# Autodesk Inventor assembly: Frame
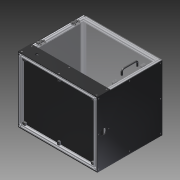
[picture p0: Inventor's stored thumbnail of the model, 180x180]
Saved by Autodesk Inventor 2015 SP1 (Build 190203100, 203)
## iProperties
Created: 2014-08-02
Part Number: Frame
Document SubType Name: Assembly
Designer: Jack
Mass: 3721.39 g
Surface Area: 12751.2 cm^2
Volume: 1360.83 cm^3
Density: 2.73465 g/cm^3
Author: Jack
Title: Frame
## Documents named in this file (29)
- C:\Users\Jack\ownCloud\Projects\CoreXY\InventorModel\Frame\Frame.iam
- C:\Users\Jack\ownCloud\Projects\CoreXY\InventorModel\Frame\FrameFrontBack.ipt
- C:\Users\Jack\ownCloud\Projects\CoreXY\InventorModel\Frame\FrameSide.ipt
- C:\Users\Jack\ownCloud\Projects\CoreXY\InventorModel\Frame\FrameUpright.ipt
- C:\Users\Jack\ownCloud\Projects\CoreXY\InventorModel\Hardware\Bolts\BlindExtrusionScrew\BlindExtrusionScrew5\M5x20BlindScrew.ipt
- C:\Users\Jack\ownCloud\Projects\CoreXY\InventorModel\Frame\FrameExtruderVerticalSupport.ipt
- C:\Users\Jack\ownCloud\Projects\CoreXY\InventorModel\Enclosure\EnclosurePanelBack.ipt
- C:\Users\Jack\ownCloud\Projects\CoreXY\InventorModel\Enclosure\EnclosurePanelBottomFront.ipt
- C:\Users\Jack\ownCloud\Projects\CoreXY\InventorModel\Enclosure\ElectronicsLowerPanel.ipt
- C:\Users\Jack\ownCloud\Projects\CoreXY\InventorModel\Enclosure\EnclosureDoorFront.ipt
- C:\Users\Jack\ownCloud\Projects\CoreXY\InventorModel\Hardware\PanelMounts\HCBR5.ipt
- C:\Users\Jack\ownCloud\Projects\CoreXY\InventorModel\Hardware\Bolts\SHCS\SHCS5\SHCS5x15.ipt
- C:\Users\Jack\ownCloud\Projects\CoreXY\InventorModel\Hardware\Hinges\HingeSHHPSK5-2\SHHPSK5_2.iam
- C:\Users\Jack\ownCloud\Projects\CoreXY\InventorModel\Hardware\FrameBrace\FrameBraceHBLFSN5-4.ipt
- C:\Users\Jack\ownCloud\Projects\CoreXY\InventorModel\Enclosure\ElectronicsTopPanel.ipt
- C:\Users\Jack\ownCloud\Projects\CoreXY\InventorModel\Hardware\Handles\HandleUWANGF100-5.ipt
- C:\Users\Jack\ownCloud\Projects\CoreXY\InventorModel\Hardware\Bolts\SHCS\SHCS4\SHCS4x10.ipt
- C:\Users\Jack\ownCloud\Projects\CoreXY\InventorModel\Hardware\Nuts\ExtrusionNuts\ExtrusionNutHNTT5-4.ipt
- C:\Users\Jack\ownCloud\Projects\CoreXY\InventorModel\Hardware\BoltWashers\BoltWasher5\BoltWasher5x8.iam
- C:\Users\Jack\ownCloud\Projects\CoreXY\InventorModel\Hardware\Nuts\Nut4.ipt
- C:\Users\Jack\ownCloud\Projects\CoreXY\InventorModel\Hardware\BoltWashers\BoltWasher5\BoltWasher5x10.iam
- C:\Users\Jack\ownCloud\Projects\CoreXY\InventorModel\Hardware\Nuts\ExtrusionNuts\ExtrusionNutLockHNTR5-4.ipt
- C:\Users\Jack\ownCloud\Projects\CoreXY\InventorModel\Hardware\Bolts\FHS\FHS4\FHS4x10.ipt
- C:\Users\Jack\ownCloud\Projects\CoreXY\InventorModel\Enclosure\EnclosurePanelLeft.ipt
- C:\Users\Jack\ownCloud\Projects\CoreXY\InventorModel\Enclosure\EnclosurePanelRight.ipt
- C:\Users\Jack\ownCloud\Projects\CoreXY\InventorModel\Hardware\Bolts\SHCS\SHCS5\SHCS5x16.ipt
- C:\Users\Jack\ownCloud\Projects\CoreXY\InventorModel\Hardware\Catches\CatchMagnetHMEN5-5\HMEN5_5_dps.ipt
- C:\Users\Jack\ownCloud\Projects\CoreXY\InventorModel\Hardware\Catches\CatchMagnetHMEN5-5\HMEN5_5_magnet.ipt
- C:\Users\Jack\ownCloud\Projects\CoreXY\InventorModel\Hardware\BoltWashers\BoltWasher4\BoltWasher4x8.iam
## Components (204 placed, 28 different names)
1. SHCS5x16:1 — Mate:400, Mate:403
2. SHCS5x16:2 — Mate:401, Mate:402
3. FrameSide:6 — Mate:66, Flush:32, Flush:33, Mate:136, Mate:146, Flush:74, Mate:148, Flush:75, Mate:181, Mate:183, Mate:211, Angle:2, Angle:21, Mate:328
4. FrameSide:5 — Mate:64, Flush:28, Flush:30, Mate:138, Mate:151, Flush:78, Mate:152, Flush:79, Mate:180, Mate:184, Mate:214, Angle:3, Angle:36, Angle:51, Mate:398
5. FrameSide:4 — Mate:52, Flush:23, Flush:25, Flush:26, Mate:84, Flush:51, Mate:86, Flush:52, Mate:94, Angle:35, Angle:50, Mate:397
6. FrameSide:3 — Mate:51, Flush:22, Flush:27, Mate:88, Flush:53, Mate:90, Flush:54, Angle:20, Mate:329
7. FrameSide:1 — Mate:1, Flush:1, Flush:2, Mate:3, Flush:5, Flush:6, Mate:18, Mate:22, Angle:25, Mate:342, Flush:114, Mate:363
8. FrameSide:2 — Mate:6, Flush:11, Flush:12, Mate:7, Mate:25, Mate:26, Mate:343, Flush:113, Angle:40, Mate:379
9. FrameExtruderVerticalSupport:1 — Mate:67, Flush:37, Mate:69, Mate:123, Flush:64, Mate:176, Mate:178, Mate:231, Angle:11
10. FrameExtruderVerticalSupport:2 — Mate:68, Flush:36, Mate:70, Mate:124, Flush:65, Mate:177, Mate:179, Mate:230, Angle:12
11. FrameUpright:1 — Mate:1, Flush:1, Flush:2, Mate:2, Flush:3, Flush:4, Mate:42, Mate:43, Mate:48, Mate:49, Mate:53, Flush:21, Flush:22, Mate:61, Mate:62, Mate:65, Mate:66, Flush:33, Flush:34, Mate:70, Flush:69, Mate:132, Mate:191, Mate:199, Mate:229, Angle:10, Angle:22, Angle:23, Angle:24, Mate:325, Mate:326, Mate:327, Angle:47, Angle:48, Angle:49, Mate:390, Mate:391, Mate:392
12. FrameUpright:2 — Mate:3, Flush:5, Flush:6, Mate:5, Flush:9, Flush:10, Mate:12, Mate:13, Mate:19, Mate:21, Mate:36, Mate:37, Mate:50, Mate:51, Mate:54, Mate:55, Mate:56, Flush:61, Mate:112, Mate:113, Mate:114, Mate:115, Mate:116, Mate:117, Mate:137, Flush:71, Mate:192, Mate:193, Mate:210, Angle:1, Angle:13, Angle:14, Angle:15, Angle:16, Mate:252, Mate:253, Mate:254, Mate:255, Mate:281, Angle:17, Angle:18, Mate:323, Angle:19, Mate:324, Angle:26, Angle:27, Mate:338, Mate:339, Flush:115
13. FrameUpright:3 — Mate:7, Mate:8, Flush:13, Mate:38, Mate:39, Mate:46, Mate:47, Mate:52, Flush:23, Flush:24, Mate:57, Mate:58, Mate:63, Mate:64, Flush:28, Flush:29, Mate:139, Flush:72, Mate:194, Mate:195, Mate:227, Angle:8, Angle:28, Angle:29, Mate:336, Mate:337, Flush:116, Mate:365, Angle:32, Mate:367, Mate:369, Angle:33, Angle:34, Mate:404, Flush:136, Mate:405, Flush:137, Mate:410, Angle:52, Mate:411, Mate:414, Angle:53, Mate:417, Mate:420, Mate:421, Mate:422, Mate:423
14. FrameUpright:4 — Mate:4, Flush:7, Flush:8, Mate:6, Flush:11, Flush:12, Mate:40, Mate:41, Mate:44, Mate:45, Mate:59, Mate:60, Mate:69, Mate:134, Flush:70, Mate:190, Mate:198, Mate:228, Angle:9, Mate:373, Angle:37, Mate:375, Angle:38, Mate:377, Angle:39, Flush:135, Mate:381, Angle:41, Angle:43, Angle:44, Mate:395, Mate:396
15. FrameFrontBack:3 — Mate:50, Flush:24, Flush:25, Mate:54, Flush:35, Flush:39, Mate:85, Mate:91, Mate:92, Flush:55, Angle:31, Mate:341
16. FrameFrontBack:6 — Mate:65, Flush:34, Mate:67, Mate:68, Flush:36, Flush:37, Mate:122, Mate:125, Mate:130, Mate:135, Mate:149, Mate:154, Mate:186, Mate:187, Mate:196, Mate:197, Mate:216, Angle:4, Mate:219, Angle:5, Mate:222, Angle:6, Mate:224, Angle:7, Angle:45, Mate:393
17. FrameFrontBack:5 — Mate:63, Flush:29, Flush:30, Flush:32, Flush:35, Mate:73, Mate:118, Mate:145, Flush:73, Mate:147, Mate:153, Mate:182, Mate:185, Angle:30, Mate:340, Mate:407
18. FrameFrontBack:4 — Mate:53, Flush:21, Flush:26, Flush:27, Flush:44, Mate:87, Mate:89, Mate:93, Flush:56, Angle:46, Mate:394
19. FrameFrontBack:1 — Mate:2, Flush:3, Flush:4, Mate:4, Flush:7, Flush:8, Mate:23, Mate:24, Mate:76, Mate:188, Mate:189, Angle:42, Mate:399
20. FrameFrontBack:2 — Mate:5, Flush:9, Flush:10, Mate:8, Flush:13, Flush:20, Mate:20, Mate:27, Flush:63, Mate:406
21. EnclosurePanelLeft:1 — Mate:342, Flush:114, Flush:115, Mate:344, Mate:353, Mate:354, Mate:355, Flush:117, Flush:118, Flush:119, Flush:120, Mate:356, Flush:121, Mate:357, Flush:122, Mate:358, Flush:123, Mate:359, Flush:124, Mate:360, Flush:125
22. EnclosurePanelRight:1 — Mate:343, Flush:113, Flush:116, Mate:345, Mate:346, Mate:347, Mate:348, Mate:349, Mate:350, Mate:351, Mate:352, Flush:126, Flush:127, Flush:128, Mate:361, Flush:129, Flush:130, Flush:131, Flush:132, Flush:133, Flush:134
23. HandleUWANGF100-5:1 — Mate:171, Mate:172, Mate:173
24. EnclosurePanelBack:1 — Mate:76, Flush:44, Mate:298, Mate:299, Mate:300, Mate:301, Mate:302, Mate:303, Mate:304, Mate:305, Flush:96, Flush:97, Flush:98, Flush:99, Flush:100, Flush:101, Flush:102, Flush:103, Mate:306, Flush:104, Flush:135
25. EnclosurePanelBottomFront:1 — Mate:73, Flush:39, Flush:61, Mate:309, Flush:107, Mate:310, Flush:108, Mate:311, Flush:109, Mate:312, Flush:110, Mate:313, Mate:314, Flush:111, Flush:112
26. EnclosureDoorFront:1 — Mate:120, Mate:121, Mate:171, Mate:172, Mate:173, Mate:174, Mate:175, Mate:264, Mate:265, Mate:266, Mate:267, Mate:268, Mate:269, Mate:270, Mate:271, Mate:400, Mate:401, Mate:402, Mate:403, Mate:408, Mate:409, Flush:138, Flush:139, Flush:140, Flush:141
27. ExtrusionNutHNTT5-4:20 — Mate:421, Mate:423
28. ExtrusionNutHNTT5-4:19 — Mate:420, Mate:422
29. BoltWasher4x8:4 [sub-assembly] — Mate:425, Tangent:4
30. BoltWasher4x8:3 [sub-assembly] — Mate:424, Tangent:3
31. HMEN5_5_dps:1 — Mate:408, Flush:139, Flush:141
32. HMEN5_5_dps:2 — Mate:409, Flush:138, Flush:140
33. BoltWasher4x8:2 [sub-assembly] — Mate:415, Mate:416, Tangent:2
34. ExtrusionNutHNTT5-4:17 — Mate:410, Angle:52, Mate:411, Mate:412
35. ExtrusionNutHNTT5-4:18 — Mate:414, Angle:53, Mate:415, Mate:417
36. HMEN5_5_magnet:2 — Mate:405, Flush:137, Mate:406, Tangent:1, Mate:413, Mate:416, Tangent:2
37. BoltWasher4x8:1 [sub-assembly] — Mate:412, Tangent:1, Mate:413
38. HMEN5_5_magnet:1 — Mate:404, Flush:136, Mate:407, Mate:424, Mate:425, Tangent:3, Tangent:4
39. ExtrusionNutLockHNTR5-4:26 — Mate:382, Angle:44, Mate:395
40. ExtrusionNutLockHNTR5-4:27 — Mate:383, Angle:43, Mate:396
41. ExtrusionNutLockHNTR5-4:28 — Mate:384, Angle:42, Mate:399
42. ExtrusionNutLockHNTR5-4:29 — Mate:385, Angle:49, Mate:390
43. ExtrusionNutLockHNTR5-4:30 — Mate:386, Angle:48, Mate:391
44. ExtrusionNutLockHNTR5-4:31 — Mate:387, Angle:47, Mate:392
45. ExtrusionNutLockHNTR5-4:32 — Mate:388, Angle:46, Mate:394
46. ExtrusionNutLockHNTR5-4:33 — Mate:389, Angle:45, Mate:393
47. ExtrusionNutLockHNTR5-4:25 — Mate:380, Mate:381, Angle:41
48. FHS4x10:22 — Mate:303, Flush:98, Mate:383
49. FHS4x10:25 — Mate:306, Flush:104, Mate:384
50. FHS4x10:23 — Mate:304, Flush:97, Mate:382
51. FHS4x10:24 — Mate:305, Flush:96, Mate:380
52. FHS4x10:21 — Mate:302, Flush:99, Mate:389
53. FHS4x10:20 — Mate:301, Flush:100, Mate:388
54. FHS4x10:19 — Mate:300, Flush:101, Mate:387
55. FHS4x10:18 — Mate:299, Flush:102, Mate:386
56. FHS4x10:17 — Mate:298, Flush:103, Mate:385
57. ExtrusionNutLockHNTR5-4:1 — Mate:281, Angle:17, Mate:362
58. ExtrusionNutLockHNTR5-4:2 — Mate:315, Angle:18, Mate:323
59. ExtrusionNutLockHNTR5-4:3 — Mate:316, Angle:19, Mate:324
60. ExtrusionNutLockHNTR5-4:4 — Mate:317, Angle:20, Mate:329
61. ExtrusionNutLockHNTR5-4:5 — Mate:318, Angle:21, Mate:328
62. ExtrusionNutLockHNTR5-4:6 — Mate:319, Angle:22, Mate:327
63. ExtrusionNutLockHNTR5-4:7 — Mate:320, Angle:23, Mate:326
64. ExtrusionNutLockHNTR5-4:8 — Mate:321, Angle:24, Mate:325
65. ExtrusionNutLockHNTR5-4:9 — Mate:322, Angle:25, Mate:363
66. FHS4x10:26 — Mate:318, Mate:360, Flush:125
67. FHS4x10:6 — Mate:316, Mate:355, Flush:120
68. FHS4x10:3 — Mate:319, Mate:358, Flush:123
69. FHS4x10:7 — Mate:320, Mate:357, Flush:122
70. FHS4x10:5 — Mate:321, Mate:356, Flush:121
71. FHS4x10:2 — Mate:322, Mate:344, Flush:117
72. FHS4x10:1 — Mate:353, Flush:118, Mate:362
73. FHS4x10:8 — Mate:315, Mate:354, Flush:119
74. FHS4x10:4 — Mate:317, Mate:359, Flush:124
75. ExtrusionNutLockHNTR5-4:16 — Mate:364, Mate:365, Angle:32
76. ExtrusionNutLockHNTR5-4:17 — Mate:366, Mate:367, Angle:34
77. ExtrusionNutLockHNTR5-4:18 — Mate:368, Mate:369, Angle:33
78. ExtrusionNutLockHNTR5-4:19 — Mate:370, Angle:35, Angle:50, Mate:397
79. ExtrusionNutLockHNTR5-4:20 — Mate:371, Angle:36, Angle:51, Mate:398
80. ExtrusionNutLockHNTR5-4:21 — Mate:372, Mate:373, Angle:37
81. ExtrusionNutLockHNTR5-4:22 — Mate:374, Mate:375, Angle:38
82. ExtrusionNutLockHNTR5-4:23 — Mate:376, Mate:377, Angle:39
83. ExtrusionNutLockHNTR5-4:24 — Mate:378, Angle:40, Mate:379
84. FHS4x10:27 — Mate:349, Flush:134, Mate:371
85. FHS4x10:14 — Mate:348, Flush:133, Mate:370
86. FHS4x10:16 — Mate:347, Flush:128, Mate:364
87. FHS4x10:11 — Mate:346, Flush:127, Mate:366
88. FHS4x10:10 — Mate:345, Flush:126, Mate:368
89. FHS4x10:9 — Mate:352, Flush:130, Mate:376
90. FHS4x10:15 — Mate:361, Flush:129, Mate:378
91. FHS4x10:12 — Mate:351, Flush:131, Mate:374
92. FHS4x10:13 — Mate:350, Flush:132, Mate:372
93. ExtrusionNutLockHNTR5-4:10 — Mate:330, Angle:27, Mate:338
94. ExtrusionNutLockHNTR5-4:11 — Mate:331, Angle:26, Mate:339
95. ExtrusionNutLockHNTR5-4:12 — Mate:332, Angle:31, Mate:341
96. ExtrusionNutLockHNTR5-4:13 — Mate:333, Angle:30, Mate:340
97. ExtrusionNutLockHNTR5-4:14 — Mate:334, Angle:28, Mate:336
98. ExtrusionNutLockHNTR5-4:15 — Mate:335, Angle:29, Mate:337
99. FHS4x10:28 — Mate:309, Flush:107, Mate:331
100. FHS4x10:29 — Mate:310, Flush:108, Mate:330
101. FHS4x10:30 — Mate:311, Flush:109, Mate:332
102. FHS4x10:31 — Mate:312, Flush:110, Mate:333
103. FHS4x10:32 — Mate:313, Flush:112, Mate:335
104. FHS4x10:33 — Mate:314, Flush:111, Mate:334
105. M5x20BlindScrew:17 — Mate:176, Mate:189
106. M5x20BlindScrew:18 — Mate:177, Mate:188
107. M5x20BlindScrew:19 — Mate:178, Mate:187
108. M5x20BlindScrew:20 — Mate:179, Mate:186
109. M5x20BlindScrew:21 — Mate:180, Mate:190
110. M5x20BlindScrew:22 — Mate:181, Mate:191
111. M5x20BlindScrew:23 — Mate:182, Mate:192
112. M5x20BlindScrew:24 — Mate:183, Mate:193
113. M5x20BlindScrew:25 — Mate:184, Mate:194
114. M5x20BlindScrew:26 — Mate:185, Mate:195
115. M5x20BlindScrew:27 — Mate:196, Mate:199
116. M5x20BlindScrew:28 — Mate:197, Mate:198
117. M5x20BlindScrew:1 — Mate:22, Mate:43
118. M5x20BlindScrew:2 — Mate:24, Mate:40
119. M5x20BlindScrew:3 — Mate:49, Mate:61
120. M5x20BlindScrew:4 — Mate:36, Mate:55
121. M5x20BlindScrew:5 — Mate:48, Mate:62
122. M5x20BlindScrew:6 — Mate:44, Mate:60
123. M5x20BlindScrew:7 — Mate:46, Mate:58
124. M5x20BlindScrew:8 — Mate:27, Mate:38
125. M5x20BlindScrew:9 — Mate:26, Mate:39
126. M5x20BlindScrew:10 — Mate:25, Mate:41
127. M5x20BlindScrew:11 — Mate:20, Mate:21
128. M5x20BlindScrew:12 — Mate:23, Mate:42
129. M5x20BlindScrew:13 — Mate:37, Mate:56
130. M5x20BlindScrew:14 — Mate:45, Mate:59
131. M5x20BlindScrew:15 — Mate:47, Mate:57
132. M5x20BlindScrew:16 — Mate:18, Mate:19
133. ExtrusionNutHNTT5-4:1 — Mate:208, Mate:211, Angle:2
134. ExtrusionNutHNTT5-4:2 — Mate:209, Mate:210, Angle:1
135. ExtrusionNutHNTT5-4:3 — Mate:212, Mate:214, Angle:3
136. ExtrusionNutHNTT5-4:4 — Mate:213, Mate:227, Angle:8
137. ExtrusionNutHNTT5-4:5 — Mate:215, Mate:216, Angle:4
138. ExtrusionNutHNTT5-4:6 — Mate:217, Mate:228, Angle:9
139. ExtrusionNutHNTT5-4:7 — Mate:218, Mate:219, Angle:5
140. ExtrusionNutHNTT5-4:8 — Mate:220, Mate:229, Angle:10
141. ExtrusionNutHNTT5-4:9 — Mate:221, Mate:222, Angle:6
142. ExtrusionNutHNTT5-4:10 — Mate:223, Mate:224, Angle:7
143. ExtrusionNutHNTT5-4:11 — Mate:225, Mate:230, Angle:12
144. ExtrusionNutHNTT5-4:12 — Mate:226, Mate:231, Angle:11
145. SHCS4x10:3 — Mate:201, Mate:202
146. SHCS4x10:12 — Mate:200, Mate:203
147. SHCS4x10:9 — Mate:232, Mate:244
148. SHCS4x10:11 — Mate:233, Mate:247
149. SHCS4x10:6 — Mate:235, Mate:243
150. SHCS4x10:8 — Mate:234, Mate:246
151. SHCS4x10:7 — Mate:236, Mate:245
152. SHCS4x10:1 — Mate:237, Mate:242
153. SHCS4x10:2 — Mate:238, Mate:241
154. SHCS4x10:5 — Mate:239, Mate:240
155. SHCS4x10:4 — Mate:205, Mate:206
156. SHCS4x10:10 — Mate:204, Mate:207
157. FrameBraceHBLFSN5-4:1 — Mate:122, Mate:123, Flush:64, Mate:223, Mate:226, Mate:236, Mate:237, Mate:242, Mate:245
158. FrameBraceHBLFSN5-4:2 — Mate:124, Flush:65, Mate:125, Mate:221, Mate:225, Mate:234, Mate:235, Mate:243, Mate:246
159. FrameBraceHBLFSN5-4:5 — Mate:130, Flush:69, Mate:132, Mate:218, Mate:220, Mate:232, Mate:233, Mate:244, Mate:247
160. FrameBraceHBLFSN5-4:7 — Mate:134, Mate:135, Flush:70, Mate:215, Mate:217, Mate:238, Mate:239, Mate:240, Mate:241
161. FrameBraceHBLFSN5-4:8 — Mate:136, Mate:137, Flush:71, Mate:200, Mate:201, Mate:202, Mate:203, Mate:208, Mate:209
162. FrameBraceHBLFSN5-4:9 — Mate:138, Mate:139, Flush:72, Mate:204, Mate:205, Mate:206, Mate:207, Mate:212, Mate:213
163. SHHPSK5_2:1 [sub-assembly] — Mate:112, Mate:113, Mate:114, Flush:63, Mate:120, Mate:174, Mate:248, Mate:249, Mate:256, Mate:257, Mate:258, Mate:259, Mate:278, Mate:279
164. SHHPSK5_2:2 [sub-assembly] — Mate:115, Mate:116, Mate:117, Mate:118, Mate:121, Mate:175, Mate:250, Mate:251, Mate:260, Mate:261, Mate:262, Mate:263, Mate:276, Mate:277
165. SHCS5x15:1 — Mate:111, Mate:142
166. SHCS5x15:2 — Mate:107, Mate:141
167. SHCS5x15:3 — Mate:108, Mate:140
168. SHCS5x15:4 — Mate:103, Mate:110, Mate:144
169. SHCS5x15:5 — Mate:104, Mate:106
170. SHCS5x15:6 — Mate:105, Mate:109, Mate:143
171. ElectronicsLowerPanel:1 — Mate:95, Mate:96, Mate:103, Mate:104, Mate:105, Mate:106, Mate:107, Mate:108, Mate:109, Mate:110, Mate:111, Mate:140, Mate:141, Mate:142
172. HCBR5:1 — Mate:84, Flush:51, Mate:85, Mate:96, Mate:144
173. HCBR5:2 — Mate:86, Flush:52, Mate:87
174. HCBR5:3 — Mate:88, Flush:53, Mate:89, Mate:95
175. HCBR5:4 — Mate:90, Flush:54, Mate:91, Mate:143
176. HCBR5:5 — Mate:92, Flush:55, Flush:57
177. HCBR5:6 — Mate:93, Flush:56, Flush:57, Mate:94
178. SHCS5x15:8 — Mate:159, Mate:165
179. SHCS5x15:10 — Mate:163, Mate:166, Mate:170
180. SHCS5x15:11 — Mate:161, Mate:168
181. SHCS5x15:12 — Mate:160, Mate:164
182. HCBR5:7 — Mate:145, Flush:73
183. HCBR5:8 — Mate:146, Flush:74, Mate:147, Mate:169
184. HCBR5:9 — Mate:148, Flush:75, Mate:149, Mate:170
185. HCBR5:11 — Mate:151, Flush:78, Mate:154, Mate:156
186. HCBR5:12 — Mate:152, Flush:79, Mate:153
187. ElectronicsTopPanel:1 — Mate:156, Mate:157, Mate:158, Mate:159, Mate:160, Mate:161, Mate:163, Mate:164, Mate:165, Mate:166, Mate:168
188. SHCS5x15:7 — Mate:157, Mate:158, Mate:169
189. BoltWasher5x10:2 [sub-assembly] — Mate:264, Mate:271, Mate:272
190. BoltWasher5x10:4 [sub-assembly] — Mate:265, Mate:270, Mate:273
191. Nut4:3 — Mate:273, Mate:278
192. Nut4:4 — Mate:272, Mate:279
193. Nut4:2 — Mate:274, Mate:277
194. BoltWasher5x10:1 [sub-assembly] — Mate:267, Mate:268, Mate:274
195. Nut4:1 — Mate:275, Mate:276
196. BoltWasher5x10:3 [sub-assembly] — Mate:266, Mate:269, Mate:275
197. BoltWasher5x8:2 [sub-assembly] — Mate:256, Mate:257
198. BoltWasher5x8:1 [sub-assembly] — Mate:258, Mate:259
199. BoltWasher5x8:4 [sub-assembly] — Mate:261, Mate:263
200. BoltWasher5x8:3 [sub-assembly] — Mate:260, Mate:262
201. ExtrusionNutHNTT5-4:13 — Mate:248, Angle:15, Mate:252
202. ExtrusionNutHNTT5-4:14 — Mate:249, Angle:16, Mate:253
203. ExtrusionNutHNTT5-4:16 — Mate:250, Angle:13, Mate:255
204. ExtrusionNutHNTT5-4:15 — Mate:251, Angle:14, Mate:254
## Relationships (517: Mate 363, Flush 97, Angle 53, Tangent 4)
- Mate:1: FrameSide:1 ↔ FrameUpright:1
- Flush:1: FrameSide:1 ↔ FrameUpright:1
- Flush:2: FrameSide:1 ↔ FrameUpright:1
- Mate:2: FrameUpright:1 ↔ FrameFrontBack:1
- Flush:3: FrameUpright:1 ↔ FrameFrontBack:1
- Flush:4: FrameUpright:1 ↔ FrameFrontBack:1
- Mate:3: FrameSide:1 ↔ FrameUpright:2
- Flush:5: FrameSide:1 ↔ FrameUpright:2
- Flush:6: FrameSide:1 ↔ FrameUpright:2
- Mate:4: FrameUpright:4 ↔ FrameFrontBack:1
- Flush:7: FrameUpright:4 ↔ FrameFrontBack:1
- Flush:8: FrameUpright:4 ↔ FrameFrontBack:1
- Mate:5: FrameUpright:2 ↔ FrameFrontBack:2
- Flush:9: FrameUpright:2 ↔ FrameFrontBack:2
- Flush:10: FrameUpright:2 ↔ FrameFrontBack:2
- Mate:6: FrameSide:2 ↔ FrameUpright:4
- Flush:11: FrameSide:2 ↔ FrameUpright:4
- Flush:12: FrameSide:2 ↔ FrameUpright:4
- Mate:7: FrameSide:2 ↔ FrameUpright:3
- Mate:8: FrameUpright:3 ↔ FrameFrontBack:2
- Flush:13: FrameUpright:3 ↔ FrameFrontBack:2
- Mate:12: FrameUpright:2
- Mate:13: FrameUpright:2
- Flush:20: FrameFrontBack:2
- Mate:18: FrameSide:1 ↔ M5x20BlindScrew:16
- Mate:19: FrameUpright:2 ↔ M5x20BlindScrew:16
- Mate:20: FrameFrontBack:2 ↔ M5x20BlindScrew:11
- Mate:21: FrameUpright:2 ↔ M5x20BlindScrew:11
- Mate:22: FrameSide:1 ↔ M5x20BlindScrew:1
- Mate:23: FrameFrontBack:1 ↔ M5x20BlindScrew:12
- Mate:24: FrameFrontBack:1 ↔ M5x20BlindScrew:2
- Mate:25: FrameSide:2 ↔ M5x20BlindScrew:10
- Mate:26: FrameSide:2 ↔ M5x20BlindScrew:9
- Mate:27: FrameFrontBack:2 ↔ M5x20BlindScrew:8
- Mate:36: FrameUpright:2 ↔ M5x20BlindScrew:4
- Mate:37: FrameUpright:2 ↔ M5x20BlindScrew:13
- Mate:38: FrameUpright:3 ↔ M5x20BlindScrew:8
- Mate:39: FrameUpright:3 ↔ M5x20BlindScrew:9
- Mate:40: FrameUpright:4 ↔ M5x20BlindScrew:2
- Mate:41: FrameUpright:4 ↔ M5x20BlindScrew:10
- Mate:42: FrameUpright:1 ↔ M5x20BlindScrew:12
- Mate:43: FrameUpright:1 ↔ M5x20BlindScrew:1
- Mate:44: FrameUpright:4 ↔ M5x20BlindScrew:6
- Mate:45: FrameUpright:4 ↔ M5x20BlindScrew:14
- Mate:46: FrameUpright:3 ↔ M5x20BlindScrew:7
- Mate:47: FrameUpright:3 ↔ M5x20BlindScrew:15
- Mate:48: FrameUpright:1 ↔ M5x20BlindScrew:5
- Mate:49: FrameUpright:1 ↔ M5x20BlindScrew:3
- Mate:50: FrameUpright:2 ↔ FrameFrontBack:3
- Mate:51: FrameSide:3 ↔ FrameUpright:2
- Mate:52: FrameSide:4 ↔ FrameUpright:3
- Mate:53: FrameUpright:1 ↔ FrameFrontBack:4
- Flush:21: FrameUpright:1 ↔ FrameFrontBack:4
- Flush:22: FrameSide:3 ↔ FrameUpright:1
- Flush:23: FrameSide:4 ↔ FrameUpright:3
- Flush:24: FrameUpright:3 ↔ FrameFrontBack:3
- Flush:25: FrameSide:4 ↔ FrameFrontBack:3
- Flush:26: FrameSide:4 ↔ FrameFrontBack:4
- Flush:27: FrameSide:3 ↔ FrameFrontBack:4
- Mate:54 (-20 mm): FrameUpright:2 ↔ FrameFrontBack:3
- Mate:55: FrameUpright:2 ↔ M5x20BlindScrew:4
- Mate:56: FrameUpright:2 ↔ M5x20BlindScrew:13
- Mate:57: FrameUpright:3 ↔ M5x20BlindScrew:15
- Mate:58: FrameUpright:3 ↔ M5x20BlindScrew:7
- Mate:59: FrameUpright:4 ↔ M5x20BlindScrew:14
- Mate:60: FrameUpright:4 ↔ M5x20BlindScrew:6
- Mate:61: FrameUpright:1 ↔ M5x20BlindScrew:3
- Mate:62: FrameUpright:1 ↔ M5x20BlindScrew:5
- Mate:63: FrameUpright:3 ↔ FrameFrontBack:5
- Mate:64: FrameSide:5 ↔ FrameUpright:3
- Flush:28: FrameSide:5 ↔ FrameUpright:3
- Flush:29: FrameUpright:3 ↔ FrameFrontBack:5
- Flush:30: FrameSide:5 ↔ FrameFrontBack:5
- [Flush]: FrameSide:6 ↔ FrameFrontBack:6
- Mate:65: FrameUpright:1 ↔ FrameFrontBack:6
- Mate:66: FrameSide:6 ↔ FrameUpright:1
- Flush:32: FrameSide:6 ↔ FrameFrontBack:5
- Flush:33: FrameSide:6 ↔ FrameUpright:1
- Flush:34: FrameUpright:1 ↔ FrameFrontBack:6
- Flush:35 (-65 mm): FrameFrontBack:3 ↔ FrameFrontBack:5
- Mate:67: FrameExtruderVerticalSupport:1 ↔ FrameFrontBack:6
- Mate:68: FrameExtruderVerticalSupport:2 ↔ FrameFrontBack:6
- Flush:36: FrameExtruderVerticalSupport:2 ↔ FrameFrontBack:6
- Flush:37: FrameExtruderVerticalSupport:1 ↔ FrameFrontBack:6
- Mate:69 (88 mm): FrameExtruderVerticalSupport:1 ↔ FrameUpright:4
- Mate:70 (88 mm): FrameExtruderVerticalSupport:2 ↔ FrameUpright:1
- Mate:73: FrameFrontBack:5 ↔ EnclosurePanelBottomFront:1
- Flush:39: FrameFrontBack:3 ↔ EnclosurePanelBottomFront:1
- Mate:76: FrameFrontBack:1 ↔ EnclosurePanelBack:1
- Flush:44: FrameFrontBack:4 ↔ EnclosurePanelBack:1
- Mate:84: FrameSide:4 ↔ HCBR5:1
- Flush:51 (3 mm): FrameSide:4 ↔ HCBR5:1
- Mate:85: FrameFrontBack:3 ↔ HCBR5:1
- Mate:86: FrameSide:4 ↔ HCBR5:2
- Flush:52 (3 mm): FrameSide:4 ↔ HCBR5:2
- Mate:87: FrameFrontBack:4 ↔ HCBR5:2
- Mate:88: FrameSide:3 ↔ HCBR5:3
- Flush:53 (3 mm): FrameSide:3 ↔ HCBR5:3
- Mate:89: FrameFrontBack:4 ↔ HCBR5:3
- Mate:90: FrameSide:3 ↔ HCBR5:4
- Flush:54 (3 mm): FrameSide:3 ↔ HCBR5:4
- Mate:91: FrameFrontBack:3 ↔ HCBR5:4
- Mate:92: FrameFrontBack:3 ↔ HCBR5:5
- Flush:55 (3 mm): FrameFrontBack:3 ↔ HCBR5:5
- Mate:93: FrameFrontBack:4 ↔ HCBR5:6
- Flush:56 (3 mm): FrameFrontBack:4 ↔ HCBR5:6
- Flush:57: HCBR5:5 ↔ HCBR5:6
- Mate:94 (225 mm): FrameSide:4 ↔ HCBR5:6
- Mate:95: ElectronicsLowerPanel:1 ↔ HCBR5:3
- Mate:96: ElectronicsLowerPanel:1 ↔ HCBR5:1
- Mate:103: SHCS5x15:4 ↔ ElectronicsLowerPanel:1
- Mate:104: SHCS5x15:5 ↔ ElectronicsLowerPanel:1
- Mate:105: SHCS5x15:6 ↔ ElectronicsLowerPanel:1
- Mate:106: SHCS5x15:5 ↔ ElectronicsLowerPanel:1
- Mate:107: SHCS5x15:2 ↔ ElectronicsLowerPanel:1
- Mate:108: SHCS5x15:3 ↔ ElectronicsLowerPanel:1
- Mate:109: SHCS5x15:6 ↔ ElectronicsLowerPanel:1
- Mate:110: SHCS5x15:4 ↔ ElectronicsLowerPanel:1
- Mate:111: SHCS5x15:1 ↔ ElectronicsLowerPanel:1
- Flush:61 (-4.7625 mm): FrameUpright:2 ↔ EnclosurePanelBottomFront:1
- Mate:112: FrameUpright:2 ↔ SHHPSK5_2:1
- Mate:113 (3 mm): FrameUpright:2 ↔ SHHPSK5_2:1
- Mate:114 (3 mm): FrameUpright:2 ↔ SHHPSK5_2:1
- Mate:115: FrameUpright:2 ↔ SHHPSK5_2:2
- Mate:116 (3 mm): FrameUpright:2 ↔ SHHPSK5_2:2
- Mate:117 (3 mm): FrameUpright:2 ↔ SHHPSK5_2:2
- Flush:63 (50 mm): FrameFrontBack:2 ↔ SHHPSK5_2:1
- Mate:118 (20 mm): FrameFrontBack:5 ↔ SHHPSK5_2:2
- Mate:120: EnclosureDoorFront:1 ↔ SHHPSK5_2:1
- Mate:121: EnclosureDoorFront:1 ↔ SHHPSK5_2:2
- Mate:122: FrameFrontBack:6 ↔ FrameBraceHBLFSN5-4:1
- Mate:123: FrameExtruderVerticalSupport:1 ↔ FrameBraceHBLFSN5-4:1
- Flush:64: FrameExtruderVerticalSupport:1 ↔ FrameBraceHBLFSN5-4:1
- Mate:124: FrameExtruderVerticalSupport:2 ↔ FrameBraceHBLFSN5-4:2
- Flush:65: FrameExtruderVerticalSupport:2 ↔ FrameBraceHBLFSN5-4:2
- Mate:125: FrameFrontBack:6 ↔ FrameBraceHBLFSN5-4:2
- Mate:130: FrameFrontBack:6 ↔ FrameBraceHBLFSN5-4:5
- Flush:69: FrameUpright:1 ↔ FrameBraceHBLFSN5-4:5
- Mate:132: FrameUpright:1 ↔ FrameBraceHBLFSN5-4:5
- Mate:134: FrameUpright:4 ↔ FrameBraceHBLFSN5-4:7
- Mate:135: FrameFrontBack:6 ↔ FrameBraceHBLFSN5-4:7
- Flush:70: FrameUpright:4 ↔ FrameBraceHBLFSN5-4:7
- Mate:136: FrameSide:6 ↔ FrameBraceHBLFSN5-4:8
- Mate:137: FrameUpright:2 ↔ FrameBraceHBLFSN5-4:8
- Flush:71: FrameUpright:2 ↔ FrameBraceHBLFSN5-4:8
- Mate:138: FrameSide:5 ↔ FrameBraceHBLFSN5-4:9
- Mate:139: FrameUpright:3 ↔ FrameBraceHBLFSN5-4:9
- Flush:72: FrameUpright:3 ↔ FrameBraceHBLFSN5-4:9
- Mate:140: SHCS5x15:3 ↔ ElectronicsLowerPanel:1
- Mate:141: SHCS5x15:2 ↔ ElectronicsLowerPanel:1
- Mate:142: SHCS5x15:1 ↔ ElectronicsLowerPanel:1
- Mate:143: SHCS5x15:6 ↔ HCBR5:4
- Mate:144: SHCS5x15:4 ↔ HCBR5:1
- Mate:145: FrameFrontBack:5 ↔ HCBR5:7
- Flush:73 (5 mm): FrameFrontBack:5 ↔ HCBR5:7
- Mate:146: FrameSide:6 ↔ HCBR5:8
- Flush:74 (5 mm): FrameSide:6 ↔ HCBR5:8
- Mate:147: FrameFrontBack:5 ↔ HCBR5:8
- Mate:148: FrameSide:6 ↔ HCBR5:9
- Flush:75 (5 mm): FrameSide:6 ↔ HCBR5:9
- Mate:149: FrameFrontBack:6 ↔ HCBR5:9
- Mate:151: FrameSide:5 ↔ HCBR5:11
- Flush:78 (5 mm): FrameSide:5 ↔ HCBR5:11
- Mate:152: FrameSide:5 ↔ HCBR5:12
- Flush:79 (5 mm): FrameSide:5 ↔ HCBR5:12
- Mate:153: FrameFrontBack:5 ↔ HCBR5:12
- Mate:154: FrameFrontBack:6 ↔ HCBR5:11
- Mate:156: HCBR5:11 ↔ ElectronicsTopPanel:1
- Mate:157: ElectronicsTopPanel:1 ↔ SHCS5x15:7
- Mate:158: ElectronicsTopPanel:1 ↔ SHCS5x15:7
- Mate:159: SHCS5x15:8 ↔ ElectronicsTopPanel:1
- Mate:160: SHCS5x15:12 ↔ ElectronicsTopPanel:1
- Mate:161: SHCS5x15:11 ↔ ElectronicsTopPanel:1
- Mate:163: SHCS5x15:10 ↔ ElectronicsTopPanel:1
- Mate:164: SHCS5x15:12 ↔ ElectronicsTopPanel:1
- Mate:165: SHCS5x15:8 ↔ ElectronicsTopPanel:1
- Mate:166: SHCS5x15:10 ↔ ElectronicsTopPanel:1
- Mate:168: SHCS5x15:11 ↔ ElectronicsTopPanel:1
- Mate:169: HCBR5:8 ↔ SHCS5x15:7
- Mate:170: SHCS5x15:10 ↔ HCBR5:9
- Mate:171: HandleUWANGF100-5:1 ↔ EnclosureDoorFront:1
- Mate:172: HandleUWANGF100-5:1 ↔ EnclosureDoorFront:1
- Mate:173: HandleUWANGF100-5:1 ↔ EnclosureDoorFront:1
- Mate:174: EnclosureDoorFront:1 ↔ SHHPSK5_2:1
- Mate:175: EnclosureDoorFront:1 ↔ SHHPSK5_2:2
- Mate:176: FrameExtruderVerticalSupport:1 ↔ M5x20BlindScrew:17
- Mate:177: FrameExtruderVerticalSupport:2 ↔ M5x20BlindScrew:18
- Mate:178: FrameExtruderVerticalSupport:1 ↔ M5x20BlindScrew:19
- Mate:179: FrameExtruderVerticalSupport:2 ↔ M5x20BlindScrew:20
- Mate:180: FrameSide:5 ↔ M5x20BlindScrew:21
- Mate:181: FrameSide:6 ↔ M5x20BlindScrew:22
- Mate:182: FrameFrontBack:5 ↔ M5x20BlindScrew:23
- Mate:183: FrameSide:6 ↔ M5x20BlindScrew:24
- Mate:184: FrameSide:5 ↔ M5x20BlindScrew:25
- Mate:185: FrameFrontBack:5 ↔ M5x20BlindScrew:26
- Mate:186: FrameFrontBack:6 ↔ M5x20BlindScrew:20
- Mate:187: FrameFrontBack:6 ↔ M5x20BlindScrew:19
- Mate:188: FrameFrontBack:1 ↔ M5x20BlindScrew:18
- Mate:189: FrameFrontBack:1 ↔ M5x20BlindScrew:17
- Mate:190: FrameUpright:4 ↔ M5x20BlindScrew:21
- Mate:191: FrameUpright:1 ↔ M5x20BlindScrew:22
- Mate:192: FrameUpright:2 ↔ M5x20BlindScrew:23
- Mate:193: FrameUpright:2 ↔ M5x20BlindScrew:24
- Mate:194: FrameUpright:3 ↔ M5x20BlindScrew:25
- Mate:195: FrameUpright:3 ↔ M5x20BlindScrew:26
- Mate:196: FrameFrontBack:6 ↔ M5x20BlindScrew:27
- Mate:197: FrameFrontBack:6 ↔ M5x20BlindScrew:28
- Mate:198: FrameUpright:4 ↔ M5x20BlindScrew:28
- Mate:199: FrameUpright:1 ↔ M5x20BlindScrew:27
- Mate:200: SHCS4x10:12 ↔ FrameBraceHBLFSN5-4:8
- Mate:201: SHCS4x10:3 ↔ FrameBraceHBLFSN5-4:8
- Mate:202: SHCS4x10:3 ↔ FrameBraceHBLFSN5-4:8
- Mate:203: SHCS4x10:12 ↔ FrameBraceHBLFSN5-4:8
- Mate:204: SHCS4x10:10 ↔ FrameBraceHBLFSN5-4:9
- Mate:205: SHCS4x10:4 ↔ FrameBraceHBLFSN5-4:9
- Mate:206: SHCS4x10:4 ↔ FrameBraceHBLFSN5-4:9
- Mate:207: SHCS4x10:10 ↔ FrameBraceHBLFSN5-4:9
- Mate:208: ExtrusionNutHNTT5-4:1 ↔ FrameBraceHBLFSN5-4:8
- Mate:209: ExtrusionNutHNTT5-4:2 ↔ FrameBraceHBLFSN5-4:8
- Mate:210: FrameUpright:2 ↔ ExtrusionNutHNTT5-4:2
- Angle:1 (0 deg): FrameUpright:2 ↔ ExtrusionNutHNTT5-4:2
- Mate:211: FrameSide:6 ↔ ExtrusionNutHNTT5-4:1
- Angle:2 (0 deg): FrameSide:6 ↔ ExtrusionNutHNTT5-4:1
- Mate:212: ExtrusionNutHNTT5-4:3 ↔ FrameBraceHBLFSN5-4:9
- Mate:213: ExtrusionNutHNTT5-4:4 ↔ FrameBraceHBLFSN5-4:9
- Mate:214: FrameSide:5 ↔ ExtrusionNutHNTT5-4:3
- Angle:3 (0 deg): FrameSide:5 ↔ ExtrusionNutHNTT5-4:3
- Mate:215: ExtrusionNutHNTT5-4:5 ↔ FrameBraceHBLFSN5-4:7
- Mate:216: FrameFrontBack:6 ↔ ExtrusionNutHNTT5-4:5
- Angle:4 (0 deg): FrameFrontBack:6 ↔ ExtrusionNutHNTT5-4:5
- Mate:217: ExtrusionNutHNTT5-4:6 ↔ FrameBraceHBLFSN5-4:7
- Mate:218: ExtrusionNutHNTT5-4:7 ↔ FrameBraceHBLFSN5-4:5
- Mate:219: FrameFrontBack:6 ↔ ExtrusionNutHNTT5-4:7
- Angle:5 (0 deg): FrameFrontBack:6 ↔ ExtrusionNutHNTT5-4:7
- Mate:220: ExtrusionNutHNTT5-4:8 ↔ FrameBraceHBLFSN5-4:5
- Mate:221: ExtrusionNutHNTT5-4:9 ↔ FrameBraceHBLFSN5-4:2
- Mate:222: FrameFrontBack:6 ↔ ExtrusionNutHNTT5-4:9
- Angle:6 (0 deg): FrameFrontBack:6 ↔ ExtrusionNutHNTT5-4:9
- Mate:223: ExtrusionNutHNTT5-4:10 ↔ FrameBraceHBLFSN5-4:1
- Mate:224: FrameFrontBack:6 ↔ ExtrusionNutHNTT5-4:10
- Angle:7 (0 deg): FrameFrontBack:6 ↔ ExtrusionNutHNTT5-4:10
- Mate:225: ExtrusionNutHNTT5-4:11 ↔ FrameBraceHBLFSN5-4:2
- Mate:226: ExtrusionNutHNTT5-4:12 ↔ FrameBraceHBLFSN5-4:1
- Mate:227: FrameUpright:3 ↔ ExtrusionNutHNTT5-4:4
- Angle:8 (0 deg): FrameUpright:3 ↔ ExtrusionNutHNTT5-4:4
- Mate:228: FrameUpright:4 ↔ ExtrusionNutHNTT5-4:6
- Angle:9 (0 deg): FrameUpright:4 ↔ ExtrusionNutHNTT5-4:6
- Mate:229: FrameUpright:1 ↔ ExtrusionNutHNTT5-4:8
- Angle:10 (0 deg): FrameUpright:1 ↔ ExtrusionNutHNTT5-4:8
- Mate:230: FrameExtruderVerticalSupport:2 ↔ ExtrusionNutHNTT5-4:11
- Mate:231: FrameExtruderVerticalSupport:1 ↔ ExtrusionNutHNTT5-4:12
- Angle:11 (0 deg): FrameExtruderVerticalSupport:1 ↔ ExtrusionNutHNTT5-4:12
- Angle:12 (0 deg): FrameExtruderVerticalSupport:2 ↔ ExtrusionNutHNTT5-4:11
- Mate:232: SHCS4x10:9 ↔ FrameBraceHBLFSN5-4:5
- Mate:233: SHCS4x10:11 ↔ FrameBraceHBLFSN5-4:5
- Mate:234: SHCS4x10:8 ↔ FrameBraceHBLFSN5-4:2
- Mate:235: SHCS4x10:6 ↔ FrameBraceHBLFSN5-4:2
- Mate:236: SHCS4x10:7 ↔ FrameBraceHBLFSN5-4:1
- Mate:237: SHCS4x10:1 ↔ FrameBraceHBLFSN5-4:1
- Mate:238: SHCS4x10:2 ↔ FrameBraceHBLFSN5-4:7
- Mate:239: SHCS4x10:5 ↔ FrameBraceHBLFSN5-4:7
- Mate:240: SHCS4x10:5 ↔ FrameBraceHBLFSN5-4:7
- Mate:241: SHCS4x10:2 ↔ FrameBraceHBLFSN5-4:7
- Mate:242: SHCS4x10:1 ↔ FrameBraceHBLFSN5-4:1
- Mate:243: SHCS4x10:6 ↔ FrameBraceHBLFSN5-4:2
- Mate:244: SHCS4x10:9 ↔ FrameBraceHBLFSN5-4:5
- Mate:245: SHCS4x10:7 ↔ FrameBraceHBLFSN5-4:1
- Mate:246: SHCS4x10:8 ↔ FrameBraceHBLFSN5-4:2
- Mate:247: SHCS4x10:11 ↔ FrameBraceHBLFSN5-4:5
- Mate:248: SHHPSK5_2:1 ↔ ExtrusionNutHNTT5-4:13
- Mate:249: SHHPSK5_2:1 ↔ ExtrusionNutHNTT5-4:14
- Mate:250: SHHPSK5_2:2 ↔ ExtrusionNutHNTT5-4:16
- Mate:251: SHHPSK5_2:2 ↔ ExtrusionNutHNTT5-4:15
- Angle:13 (0 deg): FrameUpright:2 ↔ ExtrusionNutHNTT5-4:16
- Angle:14 (0 deg): FrameUpright:2 ↔ ExtrusionNutHNTT5-4:15
- Angle:15 (0 deg): FrameUpright:2 ↔ ExtrusionNutHNTT5-4:13
- Angle:16 (0 deg): FrameUpright:2 ↔ ExtrusionNutHNTT5-4:14
- Mate:252: FrameUpright:2 ↔ ExtrusionNutHNTT5-4:13
- Mate:253: FrameUpright:2 ↔ ExtrusionNutHNTT5-4:14
- Mate:254: FrameUpright:2 ↔ ExtrusionNutHNTT5-4:15
- Mate:255: FrameUpright:2 ↔ ExtrusionNutHNTT5-4:16
- Mate:256: SHHPSK5_2:1 ↔ BoltWasher5x8:2
- Mate:257: SHHPSK5_2:1 ↔ BoltWasher5x8:2
- Mate:258: SHHPSK5_2:1 ↔ BoltWasher5x8:1
- Mate:259: SHHPSK5_2:1 ↔ BoltWasher5x8:1
- Mate:260: SHHPSK5_2:2 ↔ BoltWasher5x8:3
- Mate:261: SHHPSK5_2:2 ↔ BoltWasher5x8:4
- Mate:262: SHHPSK5_2:2 ↔ BoltWasher5x8:3
- Mate:263: SHHPSK5_2:2 ↔ BoltWasher5x8:4
- Mate:264: EnclosureDoorFront:1 ↔ BoltWasher5x10:2
- Mate:265: EnclosureDoorFront:1 ↔ BoltWasher5x10:4
- Mate:266: EnclosureDoorFront:1 ↔ BoltWasher5x10:3
- Mate:267: EnclosureDoorFront:1 ↔ BoltWasher5x10:1
- Mate:268: EnclosureDoorFront:1 ↔ BoltWasher5x10:1
- Mate:269: EnclosureDoorFront:1 ↔ BoltWasher5x10:3
- Mate:270: EnclosureDoorFront:1 ↔ BoltWasher5x10:4
- Mate:271: EnclosureDoorFront:1 ↔ BoltWasher5x10:2
- Mate:272: BoltWasher5x10:2 ↔ Nut4:4
- Mate:273: BoltWasher5x10:4 ↔ Nut4:3
- Mate:274: Nut4:2 ↔ BoltWasher5x10:1
- Mate:275: Nut4:1 ↔ BoltWasher5x10:3
- Mate:276: SHHPSK5_2:2 ↔ Nut4:1
- Mate:277: SHHPSK5_2:2 ↔ Nut4:2
- Mate:278: SHHPSK5_2:1 ↔ Nut4:3
- Mate:279: SHHPSK5_2:1 ↔ Nut4:4
- Mate:281: FrameUpright:2 ↔ ExtrusionNutLockHNTR5-4:1
- Angle:17 (180 deg): FrameUpright:2 ↔ ExtrusionNutLockHNTR5-4:1
- Mate:298: EnclosurePanelBack:1 ↔ FHS4x10:17
- Mate:299: EnclosurePanelBack:1 ↔ FHS4x10:18
- Mate:300: EnclosurePanelBack:1 ↔ FHS4x10:19
- Mate:301: EnclosurePanelBack:1 ↔ FHS4x10:20
- Mate:302: EnclosurePanelBack:1 ↔ FHS4x10:21
- Mate:303: EnclosurePanelBack:1 ↔ FHS4x10:22
- Mate:304: EnclosurePanelBack:1 ↔ FHS4x10:23
- Mate:305: EnclosurePanelBack:1 ↔ FHS4x10:24
- Flush:96: EnclosurePanelBack:1 ↔ FHS4x10:24
- Flush:97: EnclosurePanelBack:1 ↔ FHS4x10:23
- Flush:98: EnclosurePanelBack:1 ↔ FHS4x10:22
- Flush:99: EnclosurePanelBack:1 ↔ FHS4x10:21
- Flush:100: EnclosurePanelBack:1 ↔ FHS4x10:20
- Flush:101: EnclosurePanelBack:1 ↔ FHS4x10:19
- Flush:102: EnclosurePanelBack:1 ↔ FHS4x10:18
- Flush:103: EnclosurePanelBack:1 ↔ FHS4x10:17
- Mate:306: EnclosurePanelBack:1 ↔ FHS4x10:25
- Flush:104: EnclosurePanelBack:1 ↔ FHS4x10:25
- Mate:309: EnclosurePanelBottomFront:1 ↔ FHS4x10:28
- Flush:107: EnclosurePanelBottomFront:1 ↔ FHS4x10:28
- Mate:310: EnclosurePanelBottomFront:1 ↔ FHS4x10:29
- Flush:108: EnclosurePanelBottomFront:1 ↔ FHS4x10:29
- Mate:311: EnclosurePanelBottomFront:1 ↔ FHS4x10:30
- Flush:109: EnclosurePanelBottomFront:1 ↔ FHS4x10:30
- Mate:312: EnclosurePanelBottomFront:1 ↔ FHS4x10:31
- Flush:110: EnclosurePanelBottomFront:1 ↔ FHS4x10:31
- Mate:313: EnclosurePanelBottomFront:1 ↔ FHS4x10:32
- Mate:314: EnclosurePanelBottomFront:1 ↔ FHS4x10:33
- Flush:111: EnclosurePanelBottomFront:1 ↔ FHS4x10:33
- Flush:112: EnclosurePanelBottomFront:1 ↔ FHS4x10:32
- Mate:315: ExtrusionNutLockHNTR5-4:2 ↔ FHS4x10:8
- Mate:316: ExtrusionNutLockHNTR5-4:3 ↔ FHS4x10:6
- Mate:317: ExtrusionNutLockHNTR5-4:4 ↔ FHS4x10:4
- Mate:318: ExtrusionNutLockHNTR5-4:5 ↔ FHS4x10:26
- Mate:319: ExtrusionNutLockHNTR5-4:6 ↔ FHS4x10:3
- Mate:320: ExtrusionNutLockHNTR5-4:7 ↔ FHS4x10:7
- Mate:321: ExtrusionNutLockHNTR5-4:8 ↔ FHS4x10:5
- Mate:322: ExtrusionNutLockHNTR5-4:9 ↔ FHS4x10:2
- Angle:18 (180 deg): FrameUpright:2 ↔ ExtrusionNutLockHNTR5-4:2
- Mate:323: FrameUpright:2 ↔ ExtrusionNutLockHNTR5-4:2
- Angle:19 (0 deg): FrameUpright:2 ↔ ExtrusionNutLockHNTR5-4:3
- Mate:324: FrameUpright:2 ↔ ExtrusionNutLockHNTR5-4:3
- Angle:20 (0 deg): FrameSide:3 ↔ ExtrusionNutLockHNTR5-4:4
- Angle:21 (0 deg): FrameSide:6 ↔ ExtrusionNutLockHNTR5-4:5
- Angle:22 (0 deg): FrameUpright:1 ↔ ExtrusionNutLockHNTR5-4:6
- Angle:23 (0 deg): FrameUpright:1 ↔ ExtrusionNutLockHNTR5-4:7
- Angle:24 (0 deg): FrameUpright:1 ↔ ExtrusionNutLockHNTR5-4:8
- Angle:25 (0 deg): FrameSide:1 ↔ ExtrusionNutLockHNTR5-4:9
- Mate:325: FrameUpright:1 ↔ ExtrusionNutLockHNTR5-4:8
- Mate:326: FrameUpright:1 ↔ ExtrusionNutLockHNTR5-4:7
- Mate:327: FrameUpright:1 ↔ ExtrusionNutLockHNTR5-4:6
- Mate:328: FrameSide:6 ↔ ExtrusionNutLockHNTR5-4:5
- Mate:329: FrameSide:3 ↔ ExtrusionNutLockHNTR5-4:4
- Mate:330: ExtrusionNutLockHNTR5-4:10 ↔ FHS4x10:29
- Mate:331: ExtrusionNutLockHNTR5-4:11 ↔ FHS4x10:28
- Mate:332: ExtrusionNutLockHNTR5-4:12 ↔ FHS4x10:30
- Mate:333: ExtrusionNutLockHNTR5-4:13 ↔ FHS4x10:31
- Mate:334: ExtrusionNutLockHNTR5-4:14 ↔ FHS4x10:33
- Mate:335: ExtrusionNutLockHNTR5-4:15 ↔ FHS4x10:32
- Angle:26 (180 deg): FrameUpright:2 ↔ ExtrusionNutLockHNTR5-4:11
- Angle:27 (180 deg): FrameUpright:2 ↔ ExtrusionNutLockHNTR5-4:10
- Angle:28 (180 deg): FrameUpright:3 ↔ ExtrusionNutLockHNTR5-4:14
- Angle:29 (0 deg): FrameUpright:3 ↔ ExtrusionNutLockHNTR5-4:15
- Angle:30 (0 deg): FrameFrontBack:5 ↔ ExtrusionNutLockHNTR5-4:13
- Angle:31 (0 deg): FrameFrontBack:3 ↔ ExtrusionNutLockHNTR5-4:12
- Mate:336: FrameUpright:3 ↔ ExtrusionNutLockHNTR5-4:14
- Mate:337: FrameUpright:3 ↔ ExtrusionNutLockHNTR5-4:15
- Mate:338: FrameUpright:2 ↔ ExtrusionNutLockHNTR5-4:10
- Mate:339: FrameUpright:2 ↔ ExtrusionNutLockHNTR5-4:11
- Mate:340: FrameFrontBack:5 ↔ ExtrusionNutLockHNTR5-4:13
- Mate:341: FrameFrontBack:3 ↔ ExtrusionNutLockHNTR5-4:12
- Mate:342: FrameSide:1 ↔ EnclosurePanelLeft:1
- Mate:343: FrameSide:2 ↔ EnclosurePanelRight:1
- Flush:113: FrameSide:2 ↔ EnclosurePanelRight:1
- Flush:114: FrameSide:1 ↔ EnclosurePanelLeft:1
- Flush:115: FrameUpright:2 ↔ EnclosurePanelLeft:1
- Flush:116: FrameUpright:3 ↔ EnclosurePanelRight:1
- Mate:344: EnclosurePanelLeft:1 ↔ FHS4x10:2
- Mate:345: EnclosurePanelRight:1 ↔ FHS4x10:10
- Mate:346: EnclosurePanelRight:1 ↔ FHS4x10:11
- Mate:347: EnclosurePanelRight:1 ↔ FHS4x10:16
- Mate:348: EnclosurePanelRight:1 ↔ FHS4x10:14
- Mate:349: EnclosurePanelRight:1 ↔ FHS4x10:27
- Mate:350: EnclosurePanelRight:1 ↔ FHS4x10:13
- Mate:351: EnclosurePanelRight:1 ↔ FHS4x10:12
- Mate:352: EnclosurePanelRight:1 ↔ FHS4x10:9
- Mate:353: EnclosurePanelLeft:1 ↔ FHS4x10:1
- Mate:354: EnclosurePanelLeft:1 ↔ FHS4x10:8
- Mate:355: EnclosurePanelLeft:1 ↔ FHS4x10:6
- Flush:117: EnclosurePanelLeft:1 ↔ FHS4x10:2
- Flush:118: EnclosurePanelLeft:1 ↔ FHS4x10:1
- Flush:119: EnclosurePanelLeft:1 ↔ FHS4x10:8
- Flush:120: EnclosurePanelLeft:1 ↔ FHS4x10:6
- Mate:356: EnclosurePanelLeft:1 ↔ FHS4x10:5
- Flush:121: EnclosurePanelLeft:1 ↔ FHS4x10:5
- Mate:357: EnclosurePanelLeft:1 ↔ FHS4x10:7
- Flush:122: EnclosurePanelLeft:1 ↔ FHS4x10:7
- Mate:358: EnclosurePanelLeft:1 ↔ FHS4x10:3
- Flush:123: EnclosurePanelLeft:1 ↔ FHS4x10:3
- Mate:359: EnclosurePanelLeft:1 ↔ FHS4x10:4
- Flush:124: EnclosurePanelLeft:1 ↔ FHS4x10:4
- Mate:360: EnclosurePanelLeft:1 ↔ FHS4x10:26
- Flush:125: EnclosurePanelLeft:1 ↔ FHS4x10:26
- Flush:126: EnclosurePanelRight:1 ↔ FHS4x10:10
- Flush:127: EnclosurePanelRight:1 ↔ FHS4x10:11
- Flush:128: EnclosurePanelRight:1 ↔ FHS4x10:16
- Mate:361: EnclosurePanelRight:1 ↔ FHS4x10:15
- Flush:129: EnclosurePanelRight:1 ↔ FHS4x10:15
- Flush:130: EnclosurePanelRight:1 ↔ FHS4x10:9
- Flush:131: EnclosurePanelRight:1 ↔ FHS4x10:12
- Flush:132: EnclosurePanelRight:1 ↔ FHS4x10:13
- Flush:133: EnclosurePanelRight:1 ↔ FHS4x10:14
- Flush:134: EnclosurePanelRight:1 ↔ FHS4x10:27
- Mate:362: ExtrusionNutLockHNTR5-4:1 ↔ FHS4x10:1
- Mate:363: FrameSide:1 ↔ ExtrusionNutLockHNTR5-4:9
- Mate:364: ExtrusionNutLockHNTR5-4:16 ↔ FHS4x10:16
- Mate:365: FrameUpright:3 ↔ ExtrusionNutLockHNTR5-4:16
- Angle:32 (0 deg): FrameUpright:3 ↔ ExtrusionNutLockHNTR5-4:16
- Mate:366: ExtrusionNutLockHNTR5-4:17 ↔ FHS4x10:11
- Mate:367: FrameUpright:3 ↔ ExtrusionNutLockHNTR5-4:17
- Mate:368: ExtrusionNutLockHNTR5-4:18 ↔ FHS4x10:10
- Mate:369: FrameUpright:3 ↔ ExtrusionNutLockHNTR5-4:18
- Angle:33 (180 deg): FrameUpright:3 ↔ ExtrusionNutLockHNTR5-4:18
- Angle:34 (0 deg): FrameUpright:3 ↔ ExtrusionNutLockHNTR5-4:17
- Mate:370: ExtrusionNutLockHNTR5-4:19 ↔ FHS4x10:14
- Angle:35 (0 deg): FrameSide:4 ↔ ExtrusionNutLockHNTR5-4:19
- Mate:371: ExtrusionNutLockHNTR5-4:20 ↔ FHS4x10:27
- Angle:36 (0 deg): FrameSide:5 ↔ ExtrusionNutLockHNTR5-4:20
- Mate:372: ExtrusionNutLockHNTR5-4:21 ↔ FHS4x10:13
- Mate:373: FrameUpright:4 ↔ ExtrusionNutLockHNTR5-4:21
- Angle:37 (0 deg): FrameUpright:4 ↔ ExtrusionNutLockHNTR5-4:21
- Mate:374: ExtrusionNutLockHNTR5-4:22 ↔ FHS4x10:12
- Mate:375: FrameUpright:4 ↔ ExtrusionNutLockHNTR5-4:22
- Angle:38 (0 deg): FrameUpright:4 ↔ ExtrusionNutLockHNTR5-4:22
- Mate:376: ExtrusionNutLockHNTR5-4:23 ↔ FHS4x10:9
- Mate:377: FrameUpright:4 ↔ ExtrusionNutLockHNTR5-4:23
- Angle:39 (0 deg): FrameUpright:4 ↔ ExtrusionNutLockHNTR5-4:23
- Mate:378: ExtrusionNutLockHNTR5-4:24 ↔ FHS4x10:15
- Angle:40 (0 deg): FrameSide:2 ↔ ExtrusionNutLockHNTR5-4:24
- Mate:379: FrameSide:2 ↔ ExtrusionNutLockHNTR5-4:24
- Mate:380: ExtrusionNutLockHNTR5-4:25 ↔ FHS4x10:24
- Flush:135: FrameUpright:4 ↔ EnclosurePanelBack:1
- Mate:381: FrameUpright:4 ↔ ExtrusionNutLockHNTR5-4:25
- Angle:41 (0 deg): FrameUpright:4 ↔ ExtrusionNutLockHNTR5-4:25
- Mate:382: ExtrusionNutLockHNTR5-4:26 ↔ FHS4x10:23
- Mate:383: ExtrusionNutLockHNTR5-4:27 ↔ FHS4x10:22
- Mate:384: ExtrusionNutLockHNTR5-4:28 ↔ FHS4x10:25
- Mate:385: ExtrusionNutLockHNTR5-4:29 ↔ FHS4x10:17
- Mate:386: ExtrusionNutLockHNTR5-4:30 ↔ FHS4x10:18
- Mate:387: ExtrusionNutLockHNTR5-4:31 ↔ FHS4x10:19
- Mate:388: ExtrusionNutLockHNTR5-4:32 ↔ FHS4x10:20
- Mate:389: ExtrusionNutLockHNTR5-4:33 ↔ FHS4x10:21
- Angle:42 (0 deg): FrameFrontBack:1 ↔ ExtrusionNutLockHNTR5-4:28
- Angle:43 (0 deg): FrameUpright:4 ↔ ExtrusionNutLockHNTR5-4:27
- Angle:44 (0 deg): FrameUpright:4 ↔ ExtrusionNutLockHNTR5-4:26
- Angle:45 (0 deg): FrameFrontBack:6 ↔ ExtrusionNutLockHNTR5-4:33
- Angle:46 (0 deg): FrameFrontBack:4 ↔ ExtrusionNutLockHNTR5-4:32
- Angle:47 (0 deg): FrameUpright:1 ↔ ExtrusionNutLockHNTR5-4:31
- Angle:48 (0 deg): FrameUpright:1 ↔ ExtrusionNutLockHNTR5-4:30
- Angle:49 (0 deg): FrameUpright:1 ↔ ExtrusionNutLockHNTR5-4:29
- Mate:390: FrameUpright:1 ↔ ExtrusionNutLockHNTR5-4:29
- Mate:391: FrameUpright:1 ↔ ExtrusionNutLockHNTR5-4:30
- Mate:392: FrameUpright:1 ↔ ExtrusionNutLockHNTR5-4:31
- Mate:393: FrameFrontBack:6 ↔ ExtrusionNutLockHNTR5-4:33
- Mate:394: FrameFrontBack:4 ↔ ExtrusionNutLockHNTR5-4:32
- Mate:395: FrameUpright:4 ↔ ExtrusionNutLockHNTR5-4:26
- Mate:396: FrameUpright:4 ↔ ExtrusionNutLockHNTR5-4:27
- Angle:50 (0 deg): FrameSide:4 ↔ ExtrusionNutLockHNTR5-4:19
- Angle:51 (0 deg): FrameSide:5 ↔ ExtrusionNutLockHNTR5-4:20
- Mate:397: FrameSide:4 ↔ ExtrusionNutLockHNTR5-4:19
- Mate:398: FrameSide:5 ↔ ExtrusionNutLockHNTR5-4:20
- Mate:399: FrameFrontBack:1 ↔ ExtrusionNutLockHNTR5-4:28
- Mate:400: SHCS5x16:1 ↔ EnclosureDoorFront:1
- Mate:401: SHCS5x16:2 ↔ EnclosureDoorFront:1
- Mate:402: SHCS5x16:2 ↔ EnclosureDoorFront:1
- Mate:403: SHCS5x16:1 ↔ EnclosureDoorFront:1
- Mate:404: FrameUpright:3 ↔ HMEN5_5_magnet:1
- Flush:136 (5 mm): FrameUpright:3 ↔ HMEN5_5_magnet:1
- Mate:405: FrameUpright:3 ↔ HMEN5_5_magnet:2
- Flush:137 (5 mm): FrameUpright:3 ↔ HMEN5_5_magnet:2
- Mate:406 (40 mm): FrameFrontBack:2 ↔ HMEN5_5_magnet:2
- Mate:407 (40 mm): FrameFrontBack:5 ↔ HMEN5_5_magnet:1
- Mate:408: EnclosureDoorFront:1 ↔ HMEN5_5_dps:1
- Mate:409: EnclosureDoorFront:1 ↔ HMEN5_5_dps:2
- Flush:138 (30.763 mm): EnclosureDoorFront:1 ↔ HMEN5_5_dps:2
- Flush:139 (30.763 mm): EnclosureDoorFront:1 ↔ HMEN5_5_dps:1
- Flush:140 (72 mm): EnclosureDoorFront:1 ↔ HMEN5_5_dps:2
- Flush:141 (52 mm): EnclosureDoorFront:1 ↔ HMEN5_5_dps:1
- Mate:410: FrameUpright:3 ↔ ExtrusionNutHNTT5-4:17
- Angle:52 (0 deg): FrameUpright:3 ↔ ExtrusionNutHNTT5-4:17
- Mate:411 (0.1 mm): FrameUpright:3 ↔ ExtrusionNutHNTT5-4:17
- Mate:412: ExtrusionNutHNTT5-4:17 ↔ BoltWasher4x8:1
- Tangent:1 (0.1 mm): HMEN5_5_magnet:2 ↔ BoltWasher4x8:1
- Mate:413: HMEN5_5_magnet:2 ↔ BoltWasher4x8:1
- Mate:414: FrameUpright:3 ↔ ExtrusionNutHNTT5-4:18
- Angle:53 (0 deg): FrameUpright:3 ↔ ExtrusionNutHNTT5-4:18
- Mate:415: BoltWasher4x8:2 ↔ ExtrusionNutHNTT5-4:18
- Mate:416: BoltWasher4x8:2 ↔ HMEN5_5_magnet:2
- Mate:417 (0.1 mm): FrameUpright:3 ↔ ExtrusionNutHNTT5-4:18
- Tangent:2 (0.1 mm): BoltWasher4x8:2 ↔ HMEN5_5_magnet:2
- [Mate]: ExtrusionNutHNTT5-4:19 ↔ BoltWasher4x8:3
- [Mate]: ExtrusionNutHNTT5-4:20 ↔ BoltWasher4x8:4
- Mate:420: FrameUpright:3 ↔ ExtrusionNutHNTT5-4:19
- Mate:421: FrameUpright:3 ↔ ExtrusionNutHNTT5-4:20
- Mate:422 (0.1 mm): FrameUpright:3 ↔ ExtrusionNutHNTT5-4:19
- Mate:423 (0.1 mm): FrameUpright:3 ↔ ExtrusionNutHNTT5-4:20
- Mate:424: BoltWasher4x8:3 ↔ HMEN5_5_magnet:1
- Mate:425: BoltWasher4x8:4 ↔ HMEN5_5_magnet:1
- Tangent:3 (0.1 mm): BoltWasher4x8:3 ↔ HMEN5_5_magnet:1
- Tangent:4 (0.1 mm): BoltWasher4x8:4 ↔ HMEN5_5_magnet:1
## Named parameters: d167_d166 = 0 mm, d741_d732 = 0 mm, d742_d737 = 0 mm
